# Autodesk Inventor assembly: Pendolo_Inverso
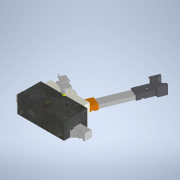
[picture p0: Inventor's stored thumbnail of the model, 180x180]
Saved by Autodesk Inventor 2020.2 (Build 242310000, 310)
## iProperties
Created: 2019-11-10
Part Number: Pendolo_Inverso
Document SubType Name: Assembly
Designer: socci
Author: socci
## Documents named in this file (12)
- C:\Users\socci\Desktop\mv-Project\04_PartDraw\Pendolo_Inverso.iam
- C:\Users\socci\Desktop\mv-Project\04_PartDraw\Componenti\19_Base_Pezzo_Unico.ipt
- C:\Users\socci\Documents\Inventor\Content Center Files\R2020\it-IT\Bearing GB_T 5800-2003\Rolling bearing GB_T 5800-2003 -635.ipt
- C:\Users\socci\Desktop\mv-Project\04_PartDraw\Componenti\1_Asse_cuscinetti.ipt
- C:\Users\socci\Desktop\mv-Project\04_PartDraw\Componenti\2_Connettore_inf_sup.ipt
- C:\Users\socci\Desktop\mv-Project\04_PartDraw\Componenti\3_Connettore_inf_INF.ipt
- C:\Users\socci\Desktop\mv-Project\04_PartDraw\Componenti\11_Connettore_MPU.ipt
- C:\Users\socci\Desktop\mv-Project\04_PartDraw\Componenti\10_MPU_6050.ipt
- C:\Users\socci\Desktop\mv-Project\04_PartDraw\Componenti\20_Base_Sopra.ipt
- C:\Users\socci\Desktop\mv-Project\04_PartDraw\Componenti\4_barra.ipt
- C:\Users\socci\Desktop\mv-Project\04_PartDraw\Componenti\8_Connettore_sup.ipt
- C:\Users\socci\Desktop\mv-Project\04_PartDraw\Componenti\22_Blocco_Escursione_Braccio.ipt
## Components (14 placed, 11 different names)
1. 19_Base_Pezzo_Unico:1 — Inserimento:1, Inserimento:2, Angolo:1, Coincidente:3, Coincidente:4, Coincidente:11, Coincidente:12, Allineato:4, Coincidente:13, Coincidente:14, Coincidente:15, Allineato:5
2. Bearing GB/T 5800-2003 635:1 — Inserimento:1, Inserimento:3, Inserimento:9
3. Bearing GB/T 5800-2003 635:2 — Inserimento:2, Inserimento:4, Inserimento:8
4. 1_Asse_cuscinetti:1 — Inserimento:3, Inserimento:4, Inserimento:5, Inserimento:6, Inserimento:7
5. 2_Connettore_inf_sup:1 — Inserimento:6, Coincidente:1, Angolo:1, Allineato:3, Coincidente:5, Coincidente:6, Coincidente:7
6. 3_Connettore_inf_INF:1 — Inserimento:5, Coincidente:1
7. 11_Connettore_MPU:1 — Coincidente:2, Allineato:1, Allineato:2, Allineato:3, Inserimento:7
8. 10_MPU_6050:1 — Coincidente:2, Allineato:1, Allineato:2
9. 20_Base_Sopra:1 — Coincidente:3, Inserimento:9
10. 20_Base_Sopra:2 — Coincidente:4, Inserimento:8
11. 4_barra:1 — Coincidente:5, Coincidente:6, Coincidente:7, Coincidente:8, Coincidente:9, Coincidente:10
12. 8_Connettore_sup:1 — Coincidente:8, Coincidente:9, Coincidente:10
13. 22_Blocco_Escursione_Braccio:1 — Coincidente:11, Coincidente:12, Allineato:4
14. 22_Blocco_Escursione_Braccio:2 — Coincidente:14, Coincidente:15, Allineato:5
## Relationships (30: Mate 15, Insert 9, Flush 5, Angle 1)
- Inserimento:1: 19_Base_Pezzo_Unico:1 ↔ Bearing GB/T 5800-2003 635:1
- Inserimento:2: 19_Base_Pezzo_Unico:1 ↔ Bearing GB/T 5800-2003 635:2
- Inserimento:3 (1.5 mm): Bearing GB/T 5800-2003 635:1 ↔ 1_Asse_cuscinetti:1
- Inserimento:4 (2.5 mm): Bearing GB/T 5800-2003 635:2 ↔ 1_Asse_cuscinetti:1
- Inserimento:5: 1_Asse_cuscinetti:1 ↔ 3_Connettore_inf_INF:1
- Inserimento:6: 1_Asse_cuscinetti:1 ↔ 2_Connettore_inf_sup:1
- Coincidente:1 [Mate] (1 mm): 2_Connettore_inf_sup:1 ↔ 3_Connettore_inf_INF:1
- Coincidente:2 [Mate] (10 mm): 11_Connettore_MPU:1 ↔ 10_MPU_6050:1
- Allineato:1 [Flush] (2 mm): 11_Connettore_MPU:1 ↔ 10_MPU_6050:1
- Allineato:2 [Flush] (3 mm): 11_Connettore_MPU:1 ↔ 10_MPU_6050:1
- Angolo:1 [Angle] (22 deg): 19_Base_Pezzo_Unico:1 ↔ 2_Connettore_inf_sup:1
- Allineato:3 [Flush] (-9.5 mm): 2_Connettore_inf_sup:1 ↔ 11_Connettore_MPU:1
- Inserimento:7: 1_Asse_cuscinetti:1 ↔ 11_Connettore_MPU:1
- Coincidente:3 [Mate] (1 mm): 19_Base_Pezzo_Unico:1 ↔ 20_Base_Sopra:1
- Coincidente:4 [Mate] (1 mm): 19_Base_Pezzo_Unico:1 ↔ 20_Base_Sopra:2
- Inserimento:8: Bearing GB/T 5800-2003 635:2 ↔ 20_Base_Sopra:2
- Inserimento:9: Bearing GB/T 5800-2003 635:1 ↔ 20_Base_Sopra:1
- Coincidente:5 [Mate] (0.5 mm): 2_Connettore_inf_sup:1 ↔ 4_barra:1
- Coincidente:6 [Mate] (0.5 mm): 2_Connettore_inf_sup:1 ↔ 4_barra:1
- Coincidente:7 [Mate]: 2_Connettore_inf_sup:1 ↔ 4_barra:1
- Coincidente:8 [Mate] (0.5 mm): 4_barra:1 ↔ 8_Connettore_sup:1
- Coincidente:9 [Mate] (0.5 mm): 4_barra:1 ↔ 8_Connettore_sup:1
- Coincidente:10 [Mate]: 4_barra:1 ↔ 8_Connettore_sup:1
- Coincidente:11 [Mate]: 19_Base_Pezzo_Unico:1 ↔ 22_Blocco_Escursione_Braccio:1
- Coincidente:12 [Mate] (0.2 mm): 19_Base_Pezzo_Unico:1 ↔ 22_Blocco_Escursione_Braccio:1
- Allineato:4 [Flush]: 19_Base_Pezzo_Unico:1 ↔ 22_Blocco_Escursione_Braccio:1
- Coincidente:13 [Mate]: 19_Base_Pezzo_Unico:1
- Coincidente:14 [Mate] (0.2 mm): 19_Base_Pezzo_Unico:1 ↔ 22_Blocco_Escursione_Braccio:2
- Coincidente:15 [Mate]: 19_Base_Pezzo_Unico:1 ↔ 22_Blocco_Escursione_Braccio:2
- Allineato:5 [Flush]: 19_Base_Pezzo_Unico:1 ↔ 22_Blocco_Escursione_Braccio:2
